# Autodesk Inventor assembly: Motor Plate Assembly
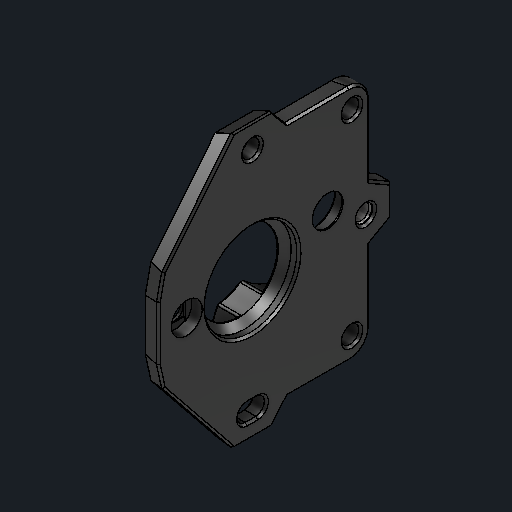
[picture p0: Inventor's stored thumbnail of the model, 512x512]
Saved by Autodesk Inventor 2026.1 (Build 301233020, 233B)
## iProperties
Created: 2025-05-11
Part Number: Motor Plate Assembly
Document SubType Name: Assembly
Designer: Joshua Eah
Author: Joshua Eah
## Documents named in this file (3)
- C:\Users\JoshuaEah\Documents\GitHub\Voron-0\CAD\Toolhead\Subassemblies\Motor Plate Assembly.iam
- C:\Users\JoshuaEah\Documents\GitHub\Voron-0\CAD\Toolhead\Parts\Toolhead Frame\Motor Plate.ipt
- C:\Users\JoshuaEah\Documents\GitHub\Voron-0\CAD\Hardware\Fasteners\M3 Hexnut.ipt
## Components (2 placed, 2 different names)
1. Motor Plate:1 — Insert:1
2. M3 Hexnut:1 — Insert:1
## Relationships (1: Insert 1)
- Insert:1: Motor Plate:1 ↔ M3 Hexnut:1
